# Autodesk Inventor assembly: neveRest+15T+pinion_MIR1
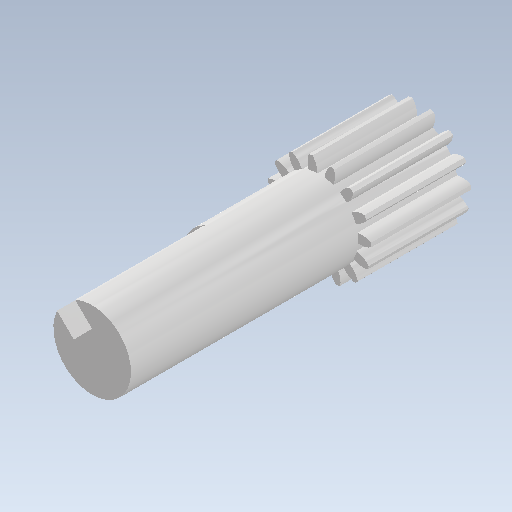
[picture p0: Inventor's stored thumbnail of the model, 512x512]
Saved by Autodesk Inventor 2020.2 (Build 242310000, 310)
## iProperties
Created: 2020-02-27
Part Number: neveRest+15T+pinion_MIR1
Document SubType Name: Assembly
Designer: deli
Author: deli
Revision Number: ANY
## Documents named in this file (3)
- C:\Users\deli\OneDrive - Eastside Preparatory School\FTC\Chassi\neveRest+15T+pinion_MIR1.iam
- C:\Users\deli\OneDrive - Eastside Preparatory School\FTC\Chassi\15T+pinion+3.2mm+bore+motor_MIR1.ipt
- C:\Users\deli\OneDrive - Eastside Preparatory School\FTC\Chassi\15T+pinion for gearbox_MIR1.ipt
## Components (2 placed, 2 different names)
1. 15T+pinion+3.2mm+bore+motor_MIR1:1 — Flush:1, Mate:2, Mate:1
2. 15T+pinion for gearbox_MIR1:1 — Flush:1, Mate:2, Mate:1
## Relationships (3: Mate 2, Flush 1)
- Flush:1: 15T+pinion+3.2mm+bore+motor_MIR1:1 ↔ 15T+pinion for gearbox_MIR1:1
- Mate:2: 15T+pinion+3.2mm+bore+motor_MIR1:1 ↔ 15T+pinion for gearbox_MIR1:1
- Mate:1: 15T+pinion+3.2mm+bore+motor_MIR1:1 ↔ 15T+pinion for gearbox_MIR1:1
